# Autodesk Inventor assembly: Jump
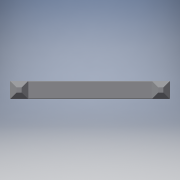
[picture p0: Inventor's stored thumbnail of the model, 180x180]
Saved by Autodesk Inventor 2016 (Build 200138000, 138)
## iProperties
Created: 2016-07-05
Part Number: Jump
Document SubType Name: Assembly
Designer: kurti
Author: kurti
## Documents named in this file (3)
- C:\Users\kurti\git\CAD\Horse Jumps\Hanging Basket Jumps\Jump.iam
- C:\Users\kurti\git\CAD\Horse Jumps\Hanging Basket Jumps\Post.ipt
- C:\Users\kurti\git\CAD\Horse Jumps\Hanging Basket Jumps\Center Support.ipt
## Components (5 placed, 2 different names)
1. Post:1 — Mate:1, Flush:1, Mate:2, Flush:2, Mate:3, Mate:4, Mate:5, Flush:3, Mate:6
2. Center Support:1 — Mate:1, Flush:1, Mate:2
3. Center Support:2 — Flush:2, Mate:3, Mate:4, Mate:7, Mate:8, Mate:9
4. Center Support:3 — Mate:5, Flush:3, Mate:6
5. Post:2 — Mate:7, Mate:8, Mate:9
## Relationships (12: Mate 9, Flush 3)
- Mate:1: Post:1 ↔ Center Support:1
- Flush:1: Post:1 ↔ Center Support:1
- Mate:2: Post:1 ↔ Center Support:1
- Flush:2: Post:1 ↔ Center Support:2
- Mate:3: Post:1 ↔ Center Support:2
- Mate:4: Post:1 ↔ Center Support:2
- Mate:5: Post:1 ↔ Center Support:3
- Flush:3: Post:1 ↔ Center Support:3
- Mate:6: Post:1 ↔ Center Support:3
- Mate:7: Center Support:2 ↔ Post:2
- Mate:8: Center Support:2 ↔ Post:2
- Mate:9: Center Support:2 ↔ Post:2
